# Autodesk Inventor assembly: vertical shooter
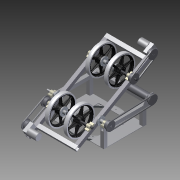
[picture p0: Inventor's stored thumbnail of the model, 180x180]
Saved by Autodesk Inventor 2011 SP1 (Build 150282100, 282)
## iProperties
Created: 2012-01-20
Part Number: vertical shooter
Document SubType Name: Assembly
Designer: Christopher
Author: Christopher
## Documents named in this file (23)
- C:\Users\Christopher\Documents\Christopher\FIRST\Inventor files\2012\shooter design 2\vertical shooter 1.2.iam
- C:\Users\Christopher\Documents\Christopher\FIRST\Inventor files\2012\shooter design 2\10 inch side piece.ipt
- C:\Users\Christopher\Documents\Christopher\FIRST\Inventor files\2011\Kit of Parts\Chassis\Chassis_Wheel_AndyMark_am-0420.iam
- C:\Users\Christopher\Documents\Christopher\FIRST\Inventor files\2012\shooter design 2\wheel hub.ipt
- C:\Users\Christopher\Documents\Christopher\FIRST\Inventor files\2012\shooter design 2\proxybearing.ipt
- C:\Users\Christopher\Documents\Christopher\FIRST\Inventor files\2012\shooter design 2\new vertical kicker thing.ipt
- C:\Users\Christopher\Documents\Christopher\FIRST\Inventor files\2012\shooter design 2\14 in axle.ipt
- C:\Users\Christopher\Documents\Christopher\FIRST\Inventor files\2012\shooter design 2\shooter 9 inch horizontal.ipt
- C:\Users\Christopher\Documents\Christopher\FIRST\Inventor files\2012\tower bottom second design\proxycimulator775.ipt
- C:\Users\Christopher\Documents\Christopher\FIRST\Inventor files\2012\4 wheel kicker version 1\proxy 775 motor.ipt
- C:\Users\Christopher\Documents\Christopher\FIRST\Inventor files\2012\tower bottom second design\2.5ingear proxy.ipt
- C:\Users\Christopher\Documents\Christopher\FIRST\Inventor files\2012\shooter design 2\shooterchain.ipt
- C:\Users\Christopher\Documents\Christopher\FIRST\Inventor files\2012\shooter design 2\new vertical kicker thingleft.ipt
- C:\Users\Christopher\Documents\Christopher\FIRST\Inventor files\2012\shooter design 2\12 inch middle piece.ipt
- C:\Users\Christopher\Documents\Christopher\FIRST\Inventor files\2012\shooter design 2\gearmotor proxy.ipt
- C:\Users\Christopher\Documents\Christopher\FIRST\Inventor files\2012\shooter design 2\gearmotor mounting plate.ipt
- C:\Users\Christopher\Documents\Christopher\FIRST\Inventor files\2012\shooter design 2\4.25 inch axle for shooter.ipt
- C:\Users\Christopher\Documents\Christopher\FIRST\Inventor files\2012\shooter design 2\shooter elevation change proxy chain.ipt
- C:\Users\Christopher\Documents\Christopher\FIRST\Inventor files\2012\shooter design 2\5 in shooter standoff.ipt
- C:\Users\Christopher\Documents\Christopher\FIRST\Inventor files\2012\tower first design\doorstop.ipt
- C:\Users\Christopher\Documents\Christopher\FIRST\Inventor files\2012\rotating turret\inner piece.ipt
- C:\Users\Christopher\Documents\Christopher\FIRST\Inventor files\2012\rotating turret\outer piece.ipt
- C:\Users\Christopher\Documents\Christopher\FIRST\Inventor files\2012\rotating turret\top plate.ipt
## Components (51 placed, 22 different names)
1. 10 inch side piece:1 — Flush:14, Flush:15, Mate:7, Mate:26, Flush:48, Flush:49, Mate:28, Flush:54, Angle:1, Mate:32, Flush:58, Flush:59, Mate:33, Flush:60
2. 10 inch side piece:2 — Mate:8, Flush:16, Flush:17, Flush:52, Flush:53, Mate:27, Flush:57, Mate:34, Flush:61, Mate:35, Flush:62, Flush:63
3. Chassis_Wheel_AndyMark_am-0420:1 [sub-assembly] — Insert:1
4. Chassis_Wheel_AndyMark_am-0420:2 [sub-assembly] — Insert:2
5. Chassis_Wheel_AndyMark_am-0420:3 [sub-assembly] — Insert:3
6. Chassis_Wheel_AndyMark_am-0420:4 [sub-assembly] — Insert:4
7. wheel hub:1 — Insert:1, Insert:10
8. wheel hub:2 — Insert:2, Insert:9
9. wheel hub:3 — Insert:3, Insert:11
10. wheel hub:4 — Insert:4, Insert:12
11. proxybearing:1 — Insert:8, Insert:17, Mate:25
12. proxybearing:2 — Mate:8, Flush:16, Flush:17, Insert:23, Insert:31
13. proxybearing:3 — Insert:7, Mate:24
14. proxybearing:4 — Mate:13, Flush:27, Insert:6, Insert:16, Mate:31
15. proxybearing:5 — Flush:14, Flush:15, Mate:7, Insert:30
16. proxybearing:6 — Mate:12, Flush:24, Insert:5, Flush:38, Mate:31
17. new vertical kicker thing:2 — Mate:12, Flush:24, Mate:13, Flush:27, Mate:16, Flush:32, Flush:33, Mate:18, Flush:36, Flush:37, Mate:20, Flush:42, Flush:43, Insert:21, Insert:24, Angle:1
18. 14 in axle:1 — Insert:6, Insert:7, Insert:11, Insert:12
19. 14 in axle:2 — Insert:5, Insert:8, Insert:9, Insert:10
20. shooter 9 inch horizontal:1 — Mate:16, Flush:32, Flush:33, Flush:38, Mate:21, Mate:22, Flush:47
21. shooter 9 inch horizontal:2 — Mate:18, Flush:36, Flush:37, Flush:44
22. proxycimulator775:1 — Insert:13, Mate:20, Flush:42, Flush:43, Insert:15
23. proxycimulator775:2 — Insert:14, Insert:18, Flush:45, Mate:23, Flush:46
24. proxy 775 motor:1 — Insert:13
25. proxy 775 motor:2 — Insert:14
26. 2.5ingear proxy:1 — Insert:15, Insert:19
27. 2.5ingear proxy:2 — Insert:16, Insert:28
28. 2.5ingear proxy:3 — Insert:18, Insert:20
29. 2.5ingear proxy:4 — Insert:17, Insert:27
30. shooterchain:1 — Insert:19, Insert:28
31. shooterchain:2 — Insert:20, Insert:27
32. new vertical kicker thingleft:1 — Mate:21, Flush:44, Mate:22, Flush:45, Mate:23, Flush:46, Flush:47, Mate:24, Mate:25, Insert:22, Insert:25, Insert:26
33. wheel hub:5 — Insert:21, Insert:24
34. wheel hub:6 — Insert:22, Insert:23, Insert:25, Insert:26
35. 12 inch middle piece:1 — Mate:26, Flush:48, Flush:49, Flush:52, Flush:53, Mate:27, Flush:55, Mate:29, Flush:56
36. gearmotor proxy:1 — Insert:29, Insert:33
37. gearmotor mounting plate:1 — Insert:29, Mate:28, Flush:54, Flush:55
38. 4.25 inch axle for shooter:1 — Insert:31
39. 4.25 inch axle for shooter:2 — Insert:30, Insert:32
40. 2.5ingear proxy:5 — Insert:32, Insert:35
41. 2.5ingear proxy:6 — Insert:33, Insert:34
42. shooter elevation change proxy chain:1 — Insert:34, Insert:35
43. 5 in shooter standoff:1 — Mate:29, Flush:56, Flush:57, Mate:30, Tangent:1, Tangent:2
44. doorstop:1 — Mate:30, Tangent:1, Tangent:2
45. 5 in shooter standoff:2 — Mate:35, Flush:62, Flush:63, Mate:36
46. 5 in shooter standoff:3 — Mate:34, Flush:61, Mate:36
47. 5 in shooter standoff:4 — Mate:33, Flush:60, Mate:37
48. 5 in shooter standoff:5 — Mate:32, Flush:58, Flush:59, Mate:37, Mate:38, Flush:64, Flush:65
49. inner piece:1 — Insert:36, Insert:37, Insert:38
50. outer piece:1 — Insert:36
51. top plate:1 — Insert:37, Insert:38, Mate:38, Flush:64, Flush:65
## Relationships (99: Insert 38, Flush 33, Mate 25, Tangent 2, Angle 1)
- Insert:1: Chassis_Wheel_AndyMark_am-0420:1 ↔ wheel hub:1
- Insert:2: Chassis_Wheel_AndyMark_am-0420:2 ↔ wheel hub:2
- Insert:3: Chassis_Wheel_AndyMark_am-0420:3 ↔ wheel hub:3
- Insert:4: Chassis_Wheel_AndyMark_am-0420:4 ↔ wheel hub:4
- Flush:14: 10 inch side piece:1 ↔ proxybearing:5
- Flush:15: 10 inch side piece:1 ↔ proxybearing:5
- Mate:7: 10 inch side piece:1 ↔ proxybearing:5
- Mate:8: 10 inch side piece:2 ↔ proxybearing:2
- Flush:16: 10 inch side piece:2 ↔ proxybearing:2
- Flush:17: 10 inch side piece:2 ↔ proxybearing:2
- Mate:12: proxybearing:6 ↔ new vertical kicker thing:2
- Flush:24: proxybearing:6 ↔ new vertical kicker thing:2
- Mate:13: proxybearing:4 ↔ new vertical kicker thing:2
- Flush:27: proxybearing:4 ↔ new vertical kicker thing:2
- Insert:5 (-12.7 mm): proxybearing:6 ↔ 14 in axle:2
- Insert:6 (-38.1 mm): proxybearing:4 ↔ 14 in axle:1
- Mate:16: new vertical kicker thing:2 ↔ shooter 9 inch horizontal:1
- Flush:32: new vertical kicker thing:2 ↔ shooter 9 inch horizontal:1
- Flush:33: new vertical kicker thing:2 ↔ shooter 9 inch horizontal:1
- Mate:18: new vertical kicker thing:2 ↔ shooter 9 inch horizontal:2
- Flush:36: new vertical kicker thing:2 ↔ shooter 9 inch horizontal:2
- Flush:37 (-63.5 mm): new vertical kicker thing:2 ↔ shooter 9 inch horizontal:2
- Flush:38 (-114.3 mm): proxybearing:6 ↔ shooter 9 inch horizontal:1
- Insert:7 (12.7 mm): proxybearing:3 ↔ 14 in axle:1
- Insert:8 (38.1 mm): proxybearing:1 ↔ 14 in axle:2
- Insert:9 (117.475 mm): wheel hub:2 ↔ 14 in axle:2
- Insert:10 (142.875 mm): wheel hub:1 ↔ 14 in axle:2
- Insert:11 (142.875 mm): wheel hub:3 ↔ 14 in axle:1
- Insert:12 (117.475 mm): wheel hub:4 ↔ 14 in axle:1
- Insert:13: proxycimulator775:1 ↔ proxy 775 motor:1
- Insert:14: proxycimulator775:2 ↔ proxy 775 motor:2
- Mate:20: new vertical kicker thing:2 ↔ proxycimulator775:1
- Flush:42: new vertical kicker thing:2 ↔ proxycimulator775:1
- Flush:43: new vertical kicker thing:2 ↔ proxycimulator775:1
- Insert:15: proxycimulator775:1 ↔ 2.5ingear proxy:1
- Insert:16: proxybearing:4 ↔ 2.5ingear proxy:2
- Insert:17: proxybearing:1 ↔ 2.5ingear proxy:4
- Insert:18: proxycimulator775:2 ↔ 2.5ingear proxy:3
- Insert:19: 2.5ingear proxy:1 ↔ shooterchain:1
- Insert:20: 2.5ingear proxy:3 ↔ shooterchain:2
- Mate:21 (63.5 mm): shooter 9 inch horizontal:1 ↔ new vertical kicker thingleft:1
- Flush:44: shooter 9 inch horizontal:2 ↔ new vertical kicker thingleft:1
- Mate:22: shooter 9 inch horizontal:1 ↔ new vertical kicker thingleft:1
- Flush:45: proxycimulator775:2 ↔ new vertical kicker thingleft:1
- Mate:23: proxycimulator775:2 ↔ new vertical kicker thingleft:1
- Flush:46: proxycimulator775:2 ↔ new vertical kicker thingleft:1
- Flush:47: shooter 9 inch horizontal:1 ↔ new vertical kicker thingleft:1
- Mate:24: proxybearing:3 ↔ new vertical kicker thingleft:1
- Mate:25: proxybearing:1 ↔ new vertical kicker thingleft:1
- Insert:21: new vertical kicker thing:2 ↔ wheel hub:5
- Insert:22: new vertical kicker thingleft:1 ↔ wheel hub:6
- Mate:26: 10 inch side piece:1 ↔ 12 inch middle piece:1
- Flush:48: 10 inch side piece:1 ↔ 12 inch middle piece:1
- Flush:49: 10 inch side piece:1 ↔ 12 inch middle piece:1
- Flush:52: 10 inch side piece:2 ↔ 12 inch middle piece:1
- Insert:23: proxybearing:2 ↔ wheel hub:6
- Flush:53: 10 inch side piece:2 ↔ 12 inch middle piece:1
- Mate:27: 10 inch side piece:2 ↔ 12 inch middle piece:1
- Insert:24: new vertical kicker thing:2 ↔ wheel hub:5
- Insert:25: new vertical kicker thingleft:1 ↔ wheel hub:6
- Insert:26: new vertical kicker thingleft:1 ↔ wheel hub:6
- Insert:27: 2.5ingear proxy:4 ↔ shooterchain:2
- Insert:28: 2.5ingear proxy:2 ↔ shooterchain:1
- Insert:29: gearmotor proxy:1 ↔ gearmotor mounting plate:1
- Mate:28: 10 inch side piece:1 ↔ gearmotor mounting plate:1
- Flush:54: 10 inch side piece:1 ↔ gearmotor mounting plate:1
- Flush:55: 12 inch middle piece:1 ↔ gearmotor mounting plate:1
- Insert:30 (-25.4 mm): proxybearing:5 ↔ 4.25 inch axle for shooter:2
- Insert:31 (-25.4 mm): proxybearing:2 ↔ 4.25 inch axle for shooter:1
- Insert:32: 4.25 inch axle for shooter:2 ↔ 2.5ingear proxy:5
- Insert:33: gearmotor proxy:1 ↔ 2.5ingear proxy:6
- Insert:34: 2.5ingear proxy:6 ↔ shooter elevation change proxy chain:1
- Insert:35: 2.5ingear proxy:5 ↔ shooter elevation change proxy chain:1
- Mate:29: 12 inch middle piece:1 ↔ 5 in shooter standoff:1
- Flush:56: 12 inch middle piece:1 ↔ 5 in shooter standoff:1
- Flush:57 (50.8 mm): 10 inch side piece:2 ↔ 5 in shooter standoff:1
- Mate:30: 5 in shooter standoff:1 ↔ doorstop:1
- Mate:31 (285.75 mm): proxybearing:4 ↔ proxybearing:6
- Angle:1 (30 deg): 10 inch side piece:1 ↔ new vertical kicker thing:2
- Mate:32: 10 inch side piece:1 ↔ 5 in shooter standoff:5
- Flush:58: 10 inch side piece:1 ↔ 5 in shooter standoff:5
- Flush:59: 10 inch side piece:1 ↔ 5 in shooter standoff:5
- Mate:33: 10 inch side piece:1 ↔ 5 in shooter standoff:4
- Flush:60: 10 inch side piece:1 ↔ 5 in shooter standoff:4
- Mate:34: 10 inch side piece:2 ↔ 5 in shooter standoff:3
- Flush:61: 10 inch side piece:2 ↔ 5 in shooter standoff:3
- Mate:35: 10 inch side piece:2 ↔ 5 in shooter standoff:2
- Flush:62: 10 inch side piece:2 ↔ 5 in shooter standoff:2
- Flush:63: 10 inch side piece:2 ↔ 5 in shooter standoff:2
- Mate:36 (254 mm): 5 in shooter standoff:2 ↔ 5 in shooter standoff:3
- Mate:37 (254 mm): 5 in shooter standoff:4 ↔ 5 in shooter standoff:5
- Insert:36: inner piece:1 ↔ outer piece:1
- Insert:37: inner piece:1 ↔ top plate:1
- Insert:38: inner piece:1 ↔ top plate:1
- Mate:38: 5 in shooter standoff:5 ↔ top plate:1
- Flush:64: 5 in shooter standoff:5 ↔ top plate:1
- Flush:65: 5 in shooter standoff:5 ↔ top plate:1
- Tangent:1 (6.35 mm): 5 in shooter standoff:1 ↔ doorstop:1
- Tangent:2 (6.35 mm): 5 in shooter standoff:1 ↔ doorstop:1
